# Autodesk Inventor assembly: complete 2nd arm
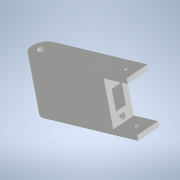
[picture p0: Inventor's stored thumbnail of the model, 180x180]
Saved by Autodesk Inventor 2022 (Build 260153000, 153)
## iProperties
Created: 2021-07-06
Part Number: complete 2nd arm
Document SubType Name: Assembly
Designer: USER
Author: USER
## Documents named in this file (4)
- F:\BVB\robotic arm\complete 2nd arm.iam
- F:\BVB\robotic arm\2nd arm.ipt
- F:\BVB\robotic arm\2nd arm closing.ipt
- F:\BVB\robotic arm\2nd to 3rd arm linking clamp.ipt
## Components (3 placed, 3 different names)
1. 2nd arm:1 — Mate:1, Flush:1, Flush:2
2. 2nd arm closing:1 — Mate:1, Flush:1, Flush:2, Mate:2, Flush:3, Flush:4
3. 2nd to 3rd arm linking clamp:1 — Mate:2, Flush:3, Flush:4
## Relationships (6: Flush 4, Mate 2)
- Mate:1: 2nd arm:1 ↔ 2nd arm closing:1
- Flush:1: 2nd arm:1 ↔ 2nd arm closing:1
- Flush:2: 2nd arm:1 ↔ 2nd arm closing:1
- Mate:2: 2nd arm closing:1 ↔ 2nd to 3rd arm linking clamp:1
- Flush:3: 2nd arm closing:1 ↔ 2nd to 3rd arm linking clamp:1
- Flush:4: 2nd arm closing:1 ↔ 2nd to 3rd arm linking clamp:1
